# Autodesk Inventor assembly: x_carryage
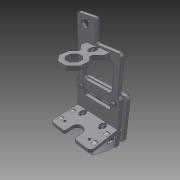
[picture p0: Inventor's stored thumbnail of the model, 180x180]
Saved by Autodesk Inventor 2014 (Build 180170000, 170)
## iProperties
Created: 2013-11-30
Part Number: x_carryage
Document SubType Name: Assembly
Designer: buben
Author: buben
## Documents named in this file (12)
- C:\Users\buben\Documents\GitHub\bacon\inventor files\assemblies\x_carryage.iam
- C:\Users\buben\Documents\GitHub\bacon\inventor files\printer parts\x_carriage_front.ipt
- C:\Users\buben\Documents\GitHub\bacon\inventor files\3rd party components\linear_bearing_8\Imported Components\LU8MM\LU8MM.iam
- C:\Users\buben\Documents\GitHub\bacon\inventor files\printer parts\x_carriage_back.ipt
- C:\Users\buben\Documents\GitHub\bacon\inventor files\utils\washer_m4.ipt
- C:\Users\buben\Documents\Inventor\Content Center Files\R2014\en-US\ISO 4762(2)\ISO 4762 - M4 x 30ISO.ipt
- C:\Users\buben\Documents\Inventor\Content Center Files\R2014\en-US\ISO 7040\ISO 7040 - M4.ipt
- C:\Users\buben\Documents\GitHub\bacon\inventor files\printer parts\x_carriage_extruder_mount.ipt
- C:\Users\buben\Documents\GitHub\bacon\inventor files\printer parts\x_carryage_brace.ipt
- C:\Users\buben\Documents\Inventor\Content Center Files\R2014\en-US\ISO 4762(2)\ISO 4762 - M4 x 35ISO.ipt
- C:\Users\buben\Documents\GitHub\bacon\inventor files\printer parts\filament_guide.ipt
- C:\Users\buben\Documents\Inventor\Content Center Files\R2014\en-US\ISO 4762(2)\ISO 4762 - M4 x 20ISO.ipt
## Components (41 placed, 11 different names)
1. x_carriage_front:1 — Mate:1, Flush:1, Flush:2, Mate:4, Mate:5, Mate:6, Mate:7, Mate:8, Mate:9, Flush:3, Mate:13, Mate:14, Mate:15, Mate:16, Mate:17, Mate:18, Mate:37, Mate:38, Flush:4, Mate:63, Mate:64, Mate:65, Mate:66, Mate:67
2. LU8MM:1 [sub-assembly] — Mate:2, Mate:3, Mate:4, Mate:5, Mate:8, Mate:10, Mate:11
3. LU8MM:2 [sub-assembly] — Mate:2, Mate:3
4. LU8MM:3 [sub-assembly] — Mate:6, Mate:7, Mate:9, Mate:12
5. x_carriage_back:1 — Mate:10, Mate:11, Mate:12, Flush:3, Mate:19, Mate:20, Mate:21, Mate:39, Mate:40, Mate:41, Mate:42, Mate:43, Mate:44, Mate:45, Mate:46
6. CSN 02 1702 B B 4,3:1 — Mate:13, Mate:18, Insert:1
7. CSN 02 1702 B B 4,3:2 — Mate:14, Mate:17, Insert:2
8. CSN 02 1702 B B 4,3:3 — Mate:15, Mate:16, Insert:3
9. ISO 4762 M4 x 30:1 — Insert:3, Mate:23, Mate:26
10. ISO 4762 M4 x 30:2 — Insert:2, Mate:22, Mate:30
11. ISO 4762 M4 x 30:3 — Insert:1, Mate:24, Mate:28
12. CSN 02 1702 B B 4,3:4 — Mate:20, Mate:23, Mate:25
13. CSN 02 1702 B B 4,3:5 — Mate:19, Mate:22, Mate:29
14. CSN 02 1702 B B 4,3:6 — Mate:21, Mate:24, Mate:27
15. DIN EN ISO 7040 M4:1 — Mate:25, Mate:26
16. DIN EN ISO 7040 M4:2 — Mate:29, Mate:30
17. DIN EN ISO 7040 M4:3 — Mate:27, Mate:28
18. x_carriage_extruder_mount:1 — Mate:31, Mate:32, Mate:33, Mate:34, Mate:35, Mate:36, Mate:37, Flush:4, Mate:49, Mate:51
19. x_carryage_brace:1 — Mate:31, Mate:34, Mate:35, Mate:38, Mate:53
20. x_carryage_brace:2 — Mate:32, Mate:33, Mate:36, Mate:47
21. CSN 02 1702 B B 4,3:7 — Mate:39, Mate:46, Insert:4
22. CSN 02 1702 B B 4,3:8 — Mate:42, Mate:43, Insert:6
23. CSN 02 1702 B B 4,3:9 — Mate:41, Mate:44, Insert:7
24. CSN 02 1702 B B 4,3:10 — Mate:40, Mate:45, Insert:5
25. ISO 4762 M4 x 35:1 — Insert:4, Mate:54, Mate:60
26. ISO 4762 M4 x 35:2 — Insert:5, Mate:52, Mate:56
27. ISO 4762 M4 x 35:3 — Insert:6, Mate:50, Mate:58
28. ISO 4762 M4 x 35:4 — Insert:7, Mate:48, Mate:62
29. CSN 02 1702 B B 4,3:11 — Mate:47, Mate:48, Mate:61
30. CSN 02 1702 B B 4,3:12 — Mate:49, Mate:50, Mate:57
31. CSN 02 1702 B B 4,3:13 — Mate:51, Mate:52, Mate:55
32. CSN 02 1702 B B 4,3:14 — Mate:53, Mate:54, Mate:59
33. DIN EN ISO 7040 M4:4 — Mate:61, Mate:62
34. DIN EN ISO 7040 M4:5 — Mate:59, Mate:60
35. DIN EN ISO 7040 M4:6 — Mate:57, Mate:58
36. DIN EN ISO 7040 M4:7 — Mate:55, Mate:56
37. filament_guide:1 — Mate:63, Mate:64, Mate:65, Mate:68
38. CSN 02 1702 B B 4,3:15 — Mate:66, Mate:67, Insert:8
39. CSN 02 1702 B B 4,3:16 — Mate:68, Mate:69, Mate:70
40. ISO 4762 M4 x 20:1 — Insert:8, Mate:69, Mate:71
41. DIN EN ISO 7040 M4:8 — Mate:70, Mate:71
## Relationships (83: Mate 71, Insert 8, Flush 4)
- Mate:1: x_carriage_front:1
- Flush:1: x_carriage_front:1
- Flush:2: x_carriage_front:1
- Mate:2: LU8MM:1 ↔ LU8MM:2
- Mate:3: LU8MM:1 ↔ LU8MM:2
- Mate:4 (7.5 mm): x_carriage_front:1 ↔ LU8MM:1
- Mate:5 (7.5 mm): x_carriage_front:1 ↔ LU8MM:1
- Mate:6 (7.5 mm): x_carriage_front:1 ↔ LU8MM:3
- Mate:7 (7.5 mm): x_carriage_front:1 ↔ LU8MM:3
- Mate:8 (0.5 mm): x_carriage_front:1 ↔ LU8MM:1
- Mate:9: x_carriage_front:1 ↔ LU8MM:3
- Mate:10 (7.5 mm): LU8MM:1 ↔ x_carriage_back:1
- Mate:11 (7.5 mm): LU8MM:1 ↔ x_carriage_back:1
- Mate:12 (7.5 mm): LU8MM:3 ↔ x_carriage_back:1
- Flush:3: x_carriage_front:1 ↔ x_carriage_back:1
- Mate:13: x_carriage_front:1 ↔ CSN 02 1702 B B 4,3:1
- Mate:14: x_carriage_front:1 ↔ CSN 02 1702 B B 4,3:2
- Mate:15: x_carriage_front:1 ↔ CSN 02 1702 B B 4,3:3
- Mate:16: x_carriage_front:1 ↔ CSN 02 1702 B B 4,3:3
- Mate:17: x_carriage_front:1 ↔ CSN 02 1702 B B 4,3:2
- Mate:18: x_carriage_front:1 ↔ CSN 02 1702 B B 4,3:1
- Insert:1: CSN 02 1702 B B 4,3:1 ↔ ISO 4762 M4 x 30:3
- Insert:2: CSN 02 1702 B B 4,3:2 ↔ ISO 4762 M4 x 30:2
- Insert:3: CSN 02 1702 B B 4,3:3 ↔ ISO 4762 M4 x 30:1
- Mate:19: x_carriage_back:1 ↔ CSN 02 1702 B B 4,3:5
- Mate:20: x_carriage_back:1 ↔ CSN 02 1702 B B 4,3:4
- Mate:21: x_carriage_back:1 ↔ CSN 02 1702 B B 4,3:6
- Mate:22: ISO 4762 M4 x 30:2 ↔ CSN 02 1702 B B 4,3:5
- Mate:23: ISO 4762 M4 x 30:1 ↔ CSN 02 1702 B B 4,3:4
- Mate:24: ISO 4762 M4 x 30:3 ↔ CSN 02 1702 B B 4,3:6
- Mate:25: CSN 02 1702 B B 4,3:4 ↔ DIN EN ISO 7040 M4:1
- Mate:26: ISO 4762 M4 x 30:1 ↔ DIN EN ISO 7040 M4:1
- Mate:27: CSN 02 1702 B B 4,3:6 ↔ DIN EN ISO 7040 M4:3
- Mate:28: ISO 4762 M4 x 30:3 ↔ DIN EN ISO 7040 M4:3
- Mate:29: CSN 02 1702 B B 4,3:5 ↔ DIN EN ISO 7040 M4:2
- Mate:30: ISO 4762 M4 x 30:2 ↔ DIN EN ISO 7040 M4:2
- Mate:31: x_carriage_extruder_mount:1 ↔ x_carryage_brace:1
- Mate:32: x_carriage_extruder_mount:1 ↔ x_carryage_brace:2
- Mate:33: x_carriage_extruder_mount:1 ↔ x_carryage_brace:2
- Mate:34: x_carriage_extruder_mount:1 ↔ x_carryage_brace:1
- Mate:35: x_carriage_extruder_mount:1 ↔ x_carryage_brace:1
- Mate:36: x_carriage_extruder_mount:1 ↔ x_carryage_brace:2
- Mate:37: x_carriage_front:1 ↔ x_carriage_extruder_mount:1
- Mate:38: x_carriage_front:1 ↔ x_carryage_brace:1
- Flush:4: x_carriage_front:1 ↔ x_carriage_extruder_mount:1
- Mate:39: x_carriage_back:1 ↔ CSN 02 1702 B B 4,3:7
- Mate:40: x_carriage_back:1 ↔ CSN 02 1702 B B 4,3:10
- Mate:41: x_carriage_back:1 ↔ CSN 02 1702 B B 4,3:9
- Mate:42: x_carriage_back:1 ↔ CSN 02 1702 B B 4,3:8
- Mate:43: x_carriage_back:1 ↔ CSN 02 1702 B B 4,3:8
- Mate:44: x_carriage_back:1 ↔ CSN 02 1702 B B 4,3:9
- Mate:45: x_carriage_back:1 ↔ CSN 02 1702 B B 4,3:10
- Mate:46: x_carriage_back:1 ↔ CSN 02 1702 B B 4,3:7
- Insert:4: CSN 02 1702 B B 4,3:7 ↔ ISO 4762 M4 x 35:1
- Insert:5: CSN 02 1702 B B 4,3:10 ↔ ISO 4762 M4 x 35:2
- Insert:6: CSN 02 1702 B B 4,3:8 ↔ ISO 4762 M4 x 35:3
- Insert:7: CSN 02 1702 B B 4,3:9 ↔ ISO 4762 M4 x 35:4
- Mate:47: x_carryage_brace:2 ↔ CSN 02 1702 B B 4,3:11
- Mate:48: ISO 4762 M4 x 35:4 ↔ CSN 02 1702 B B 4,3:11
- Mate:49: x_carriage_extruder_mount:1 ↔ CSN 02 1702 B B 4,3:12
- Mate:50: ISO 4762 M4 x 35:3 ↔ CSN 02 1702 B B 4,3:12
- Mate:51: x_carriage_extruder_mount:1 ↔ CSN 02 1702 B B 4,3:13
- Mate:52: ISO 4762 M4 x 35:2 ↔ CSN 02 1702 B B 4,3:13
- Mate:53: x_carryage_brace:1 ↔ CSN 02 1702 B B 4,3:14
- Mate:54: ISO 4762 M4 x 35:1 ↔ CSN 02 1702 B B 4,3:14
- Mate:55: CSN 02 1702 B B 4,3:13 ↔ DIN EN ISO 7040 M4:7
- Mate:56: ISO 4762 M4 x 35:2 ↔ DIN EN ISO 7040 M4:7
- Mate:57: CSN 02 1702 B B 4,3:12 ↔ DIN EN ISO 7040 M4:6
- Mate:58: ISO 4762 M4 x 35:3 ↔ DIN EN ISO 7040 M4:6
- Mate:59: CSN 02 1702 B B 4,3:14 ↔ DIN EN ISO 7040 M4:5
- Mate:60: ISO 4762 M4 x 35:1 ↔ DIN EN ISO 7040 M4:5
- Mate:61: CSN 02 1702 B B 4,3:11 ↔ DIN EN ISO 7040 M4:4
- Mate:62: ISO 4762 M4 x 35:4 ↔ DIN EN ISO 7040 M4:4
- Mate:63: x_carriage_front:1 ↔ filament_guide:1
- Mate:64: x_carriage_front:1 ↔ filament_guide:1
- Mate:65: x_carriage_front:1 ↔ filament_guide:1
- Mate:66: x_carriage_front:1 ↔ CSN 02 1702 B B 4,3:15
- Mate:67: x_carriage_front:1 ↔ CSN 02 1702 B B 4,3:15
- Insert:8: CSN 02 1702 B B 4,3:15 ↔ ISO 4762 M4 x 20:1
- Mate:68: filament_guide:1 ↔ CSN 02 1702 B B 4,3:16
- Mate:69: CSN 02 1702 B B 4,3:16 ↔ ISO 4762 M4 x 20:1
- Mate:70: CSN 02 1702 B B 4,3:16 ↔ DIN EN ISO 7040 M4:8
- Mate:71: ISO 4762 M4 x 20:1 ↔ DIN EN ISO 7040 M4:8
